# Autodesk Inventor assembly: Laeufer
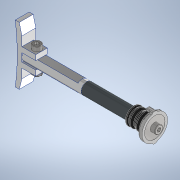
[picture p0: Inventor's stored thumbnail of the model, 180x180]
Saved by Autodesk Inventor 2021 (Build 250183000, 183)
## iProperties
Created: 2022-08-23
Part Number: Laeufer
Document SubType Name: Assembly
Designer: Timo
Author: Timo
## Documents named in this file (10)
- D:\X260_Dokumente\Soccer\hardware\Originalkicker Bangkok\Laeufer.iam
- D:\X260_Dokumente\Soccer\hardware\Originalkicker Bangkok\Shaft.ipt
- D:\X260_Dokumente\Soccer\hardware\Originalkicker Bangkok\Bolzen.ipt
- D:\X260_Dokumente\Soccer\hardware\Originalkicker Bangkok\Schaufel.ipt
- C:\Users\Timo\Documents\Inventor\Content Center Files\R2021\de-DE\AS 1420\AS 1420 - 1973 - M4 x 8.ipt
- C:\Users\Timo\Documents\Inventor\Content Center Files\R2021\de-DE\AS 1420\AS 1420 - 1973 - M4 x 20.ipt
- D:\X260_Dokumente\Soccer\hardware\Originalkicker Bangkok\Dämpfer.ipt
- D:\X260_Dokumente\Soccer\hardware\Originalkicker Bangkok\Gummibandhalter.ipt
- C:\Users\Timo\Documents\Inventor\Content Center Files\R2021\de-DE\DIN 9021\DIN 9021 - 6,4.ipt
- C:\Users\Timo\Documents\Inventor\Content Center Files\R2021\de-DE\AS 1474(1)\AS 1474 - M4(1).ipt
## Components (9 placed, 9 different names)
1. Shaft:1 — Fluchtend:1, Fluchtend:2, Fluchtend:3, Passend:1, Passend:2, Passend:3, Passend:4, Passend:5, Passend:6, Passend:9, Passend:10
2. Bolzen:1 — Passend:1, Passend:2, Passend:3, Passend:7, Passend:8
3. Schaufel:1 — Passend:4, Passend:5, Passend:6, Einfügen:1, Passend:16
4. AS 1420 - Metrisch M4 x 20:1 — Einfügen:1, Passend:15
5. Dämpfer:1 — Passend:7, Passend:8, Fluchtend:4
6. Gummibandhalter:1 — Fluchtend:4, Passend:9, Passend:10, Passend:11, Passend:12
7. DIN 9021 6,4:1 — Passend:11, Passend:12, Passend:13, Passend:14
8. AS 1420 - Metrisch M4 x 8:1 — Passend:13, Passend:14
9. AS 1474 - Metrisch M4:1 — Passend:15, Passend:16
## Relationships (21: Mate 16, Flush 4, Insert 1)
- Fluchtend:1 [Flush]: Shaft:1
- Fluchtend:2 [Flush]: Shaft:1
- Fluchtend:3 [Flush]: Shaft:1
- Passend:1 [Mate]: Shaft:1 ↔ Bolzen:1
- Passend:2 [Mate]: Shaft:1 ↔ Bolzen:1
- Passend:3 [Mate]: Shaft:1 ↔ Bolzen:1
- Passend:4 [Mate]: Shaft:1 ↔ Schaufel:1
- Passend:5 [Mate]: Shaft:1 ↔ Schaufel:1
- Passend:6 [Mate]: Shaft:1 ↔ Schaufel:1
- Einfügen:1 [Insert]: Schaufel:1 ↔ AS 1420 - Metrisch M4 x 20:1
- Passend:7 [Mate]: Bolzen:1 ↔ Dämpfer:1
- Passend:8 [Mate]: Bolzen:1 ↔ Dämpfer:1
- Fluchtend:4 [Flush]: Dämpfer:1 ↔ Gummibandhalter:1
- Passend:9 [Mate]: Shaft:1 ↔ Gummibandhalter:1
- Passend:10 [Mate]: Shaft:1 ↔ Gummibandhalter:1
- Passend:11 [Mate]: Gummibandhalter:1 ↔ DIN 9021 6,4:1
- Passend:12 [Mate]: Gummibandhalter:1 ↔ DIN 9021 6,4:1
- Passend:13 [Mate]: DIN 9021 6,4:1 ↔ AS 1420 - Metrisch M4 x 8:1
- Passend:14 [Mate]: DIN 9021 6,4:1 ↔ AS 1420 - Metrisch M4 x 8:1
- Passend:15 [Mate]: AS 1420 - Metrisch M4 x 20:1 ↔ AS 1474 - Metrisch M4:1
- Passend:16 [Mate]: Schaufel:1 ↔ AS 1474 - Metrisch M4:1
